# Autodesk Inventor assembly: frame
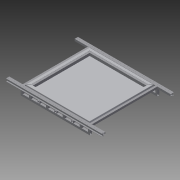
[picture p0: Inventor's stored thumbnail of the model, 180x180]
Saved by Autodesk Inventor 2013 (Build 170138000, 138)
## iProperties
Created: 2012-10-19
Part Number: frame
Document SubType Name: Assembly
Designer: Istvan
Author: Istvan
## Documents named in this file (7)
- C:\Users\istvan.burbank\Documents\GitHub\Crown-Fire\CAD\Frame\frame.iam
- C:\Users\istvan.burbank\Documents\GitHub\Crown-Fire\CAD\Frame\Table\table.iam
- C:\Users\istvan.burbank\Documents\GitHub\Crown-Fire\CAD\Frame\Supports\supports.iam
- C:\Users\istvan.burbank\Documents\GitHub\Crown-Fire\CAD\Frame\WorkTable\workTable.ipt
- C:\Users\istvan.burbank\Documents\GitHub\Crown-Fire\CAD\Frame\Gantry\y-axisTrucks\rack.ipt
- C:\Users\istvan.burbank\Documents\GitHub\Crown-Fire\CAD\Frame\GantryMount\cChannel.ipt
- C:\Users\istvan.burbank\Documents\GitHub\Crown-Fire\CAD\Templates\cChannel2x1.ipt
## Components (7 placed, 5 different names)
1. table:1 [sub-assembly] — Mate:1, Mate:2, Mate:5, Mate:6
2. supports:1 [sub-assembly] — Mate:1, Mate:2, Mate:3, Mate:4, Mate:5, Mate:6, Mate:7, Mate:8, Flush:1, Flush:2, Flush:3, Flush:4
3. workTable:1 — Mate:3, Mate:4
4. rack:1 — Mate:10, Flush:5
5. rack:2 — Mate:9, Flush:6
6. cChannel:1 — Mate:8, Flush:2, Flush:4, Mate:10, Flush:5
7. cChannel:2 — Mate:7, Flush:1, Flush:3, Mate:9, Flush:6
## Relationships (16: Mate 10, Flush 6)
- Mate:1 (12.7 mm): table:1 ↔ supports:1
- Mate:2 (12.7 mm): table:1 ↔ supports:1
- Mate:3: supports:1 ↔ workTable:1
- Mate:4: supports:1 ↔ workTable:1
- Mate:5: table:1 ↔ supports:1
- Mate:6 (6.35 mm): table:1 ↔ supports:1
- Mate:7: supports:1 ↔ cChannel:2
- Mate:8: supports:1 ↔ cChannel:1
- Flush:1: supports:1 ↔ cChannel:2
- Flush:2: supports:1 ↔ cChannel:1
- Flush:3: supports:1 ↔ cChannel:2
- Flush:4: supports:1 ↔ cChannel:1
- Mate:9: rack:2 ↔ cChannel:2
- Mate:10: rack:1 ↔ cChannel:1
- Flush:5: rack:1 ↔ cChannel:1
- Flush:6: rack:2 ↔ cChannel:2
